# Autodesk Inventor assembly: BostonDM
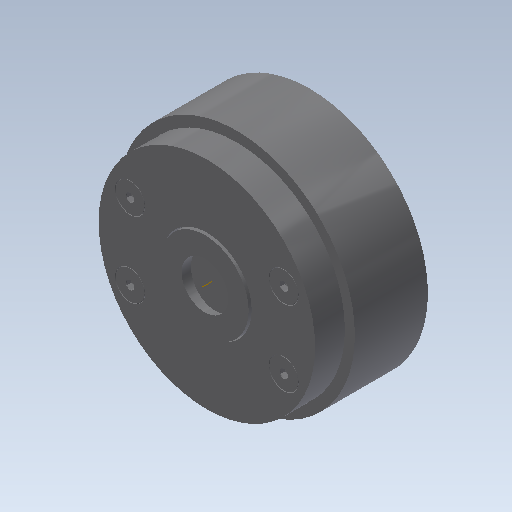
[picture p0: Inventor's stored thumbnail of the model, 512x512]
Saved by Autodesk Inventor 2020 (Build 240168000, 168)
## iProperties
Created: 2013-02-15
Part Number: BostonDM
Document SubType Name: Assembly
Designer: map
Sending System: SolidWorks 2015
Last Author: yl862
Last Saved: 2016-08-03
Author: map
## Documents named in this file (5)
- C:\Users\whgu0532\Documents\4Pi\4Pi-Oxford\BostonDM.iam
- C:\Users\whgu0532\Documents\4Pi\4Pi-Oxford\BostonDM\91253A104 (McMaster-Carr)1.ipt
- C:\Users\whgu0532\Documents\4Pi\4Pi-Oxford\BostonDM\H0120FRT0A-1.ipt
- C:\Users\whgu0532\Documents\4Pi\4Pi-Oxford\BostonDM\H0120HSG0A-2.ipt
- C:\Users\whgu0532\Documents\4Pi\4Pi-Oxford\BostonDM\B0120INF0A-1.iam
## Components (7 placed, 4 different names)
1. 91253A104 (McMaster-Carr)1:1
2. 91253A104 (McMaster-Carr)1:2
3. H0120FRT0A-1:1
4. 91253A104 (McMaster-Carr)1:3
5. H0120HSG0A-2:1
6. 91253A104 (McMaster-Carr)1:4
7. B0120INF0A-1:1 [sub-assembly] — Mate:1, Mate:2
## Relationships (3: Mate 3)
- Mate:1: B0120INF0A-1:1
- Mate:2: B0120INF0A-1:1
- Mate:3
